# Autodesk Inventor assembly: A-01-0
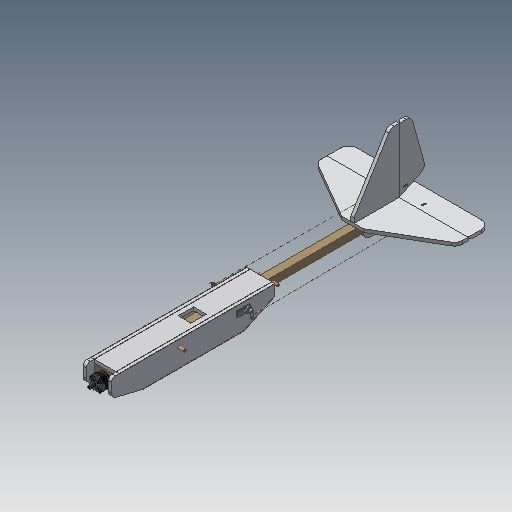
[picture p0: Inventor's stored thumbnail of the model, 512x512]
Saved by Autodesk Inventor 2019 (Build 230136000, 136)
## iProperties
Created: 2022-04-10
Part Number: A-01-0
Document SubType Name: Assembly
Designer: solyo
Mass: 82.8117 g
Surface Area: 1871.67 cm^2
Volume: 370.751 cm^3
Density: 0.223362 g/cm^3
Author: solyo
## Documents named in this file (19)
- D:\Modelling\RC\RC Trainer V1\ASSEMBLY\A-01-0-FUSELAGE\A-01-0.iam
- D:\Modelling\RC\RC Trainer V1\Parts\PW-00-0-TAILBOOM\PW-00-0-0.ipt
- D:\Modelling\RC\RC Trainer V1\Parts\PW-01-0-FIREWALL\PW-01-0-0.ipt
- D:\Modelling\RC\RC Trainer V1\Parts\PW-02-0-PIN\PW-02-0-0\WING_FRONT_TIE.ipt
- D:\Modelling\RC\RC Trainer V1\Design\Parts\PW-02-0-PIN\PW-02-0-0.ipt
- D:\Modelling\RC\RC Trainer V1\Parts\PW-02-0-PIN\PW-02-0-0\WING_REAR_TIE.ipt
- D:\Modelling\RC\RC Trainer V1\Parts\PF-01-0-FUSELAGE\PF-01-0-1.ipt
- D:\Modelling\RC\RC Trainer V1\Parts\C-01-0-EMAX_MT1806_2280KV\C-01-0.ipt
- D:\Modelling\RC\RC Trainer V1\Parts\PF-02-0-HORIZONTAL_STABILIZER\PF-02-0-0.ipt
- D:\Modelling\RC\RC Trainer V1\Parts\PF-03-0-VERTICAL_STABILIZER\PF-03-0-0.ipt
- D:\Modelling\RC\RC Trainer V1\Parts\PW-02-0-PIN\PW-02-0-0\SLIDE.ipt
- D:\Modelling\RC\RC Trainer V1\Parts\PM-00-0-PUSHROD\PM-00-0-0\TAIL.ipt
- D:\Modelling\RC\RC Trainer V1\Design\Parts\PM-00-0-PUSHROD\PM-00-0-0.ipt
- D:\Modelling\RC\RC Trainer V1\Parts\PP-00-0-CONTROL_HORN\PP-00-0-0.ipt
- D:\Modelling\RC\RC Trainer V1\Parts\C-02-0-EMAX_12AESC\C-02-0.ipt
- D:\Modelling\RC\RC Trainer V1\Parts\C-03-0-SERVO_3G\C-03-0\CW.ipt
- D:\Modelling\RC\RC Trainer V1\Design\Parts\C-03-0-SERVO_3G\C-03-0.ipt
- D:\Modelling\RC\RC Trainer V1\Parts\C-04-0-SERVO_LINKAGE_STOPPER\C-04-0.ipt
- D:\Modelling\RC\RC Trainer V1\Parts\C-05-0-FS2A_4CH\C-05-0.ipt
## Components (19 placed, 15 different names)
1. C-05-0:1 — Mate:39, Mate:40, Mate:41
2. PW-00-0-0:1
3. WING_FRONT_TIE:1
4. WING_REAR_TIE:2
5. C-02-0:1 — Mate:37, Flush:4, Mate:38
6. PW-01-0-0:1 — Flush:4, Mate:38, Mate:41
7. PF-01-0-1:1 — Flush:3, Mate:37, Mate:39, Mate:40
8. C-01-0:1
9. CW:1
10. CW:2
11. SLIDE:3
12. PF-02-0-0:1
13. PF-03-0-0:1
14. TAIL:1
15. TAIL:2
16. PP-00-0-0:1
17. PP-00-0-0:2
18. C-04-0:1
19. C-04-0:2
## Relationships (46: Mate 37, Insert 5, Flush 4)
- [Mate]: PW-00-0-0:1 ↔ PW-01-0-0:1
- [Flush]: PW-00-0-0:1 ↔ PW-01-0-0:1
- [Mate]: PW-00-0-0:1 ↔ PF-01-0-1:1
- [Mate]: PW-01-0-0:1 ↔ PF-01-0-1:1
- [Insert]: PW-01-0-0:1 ↔ C-01-0:1
- [Mate]: PW-01-0-0:1 ↔ C-01-0:1
- [Mate]: PF-02-0-0:1 ↔ PF-03-0-0:1
- [Mate]: PF-02-0-0:1 ↔ PF-03-0-0:1
- [Mate]: PF-02-0-0:1 ↔ PF-03-0-0:1
- [Mate]: PW-00-0-0:1 ↔ PF-03-0-0:1
- [Mate]: PW-00-0-0:1 ↔ PF-02-0-0:1
- [Mate]: PW-00-0-0:1 ↔ PF-03-0-0:1
- [Mate] (-2.5 mm): SLIDE:3 ↔ PF-03-0-0:1
- [Flush]: SLIDE:3 ↔ PF-03-0-0:1
- [Mate]: PF-02-0-0:1 ↔ PP-00-0-0:1
- [Mate]: PF-02-0-0:1 ↔ PP-00-0-0:1
- [Mate]: PF-03-0-0:1 ↔ PP-00-0-0:2
- [Mate]: PF-03-0-0:1 ↔ PP-00-0-0:2
- [Mate]: PW-00-0-0:1 ↔ CW:1
- [Mate]: PF-01-0-1:1 ↔ CW:1
- [Mate]: PW-00-0-0:1 ↔ CW:2
- [Mate]: PF-01-0-1:1 ↔ CW:2
- [Mate]: PF-01-0-1:1 ↔ CW:2
- [Mate] (10 mm): PF-02-0-0:1 ↔ PP-00-0-0:2
- [Mate]: PF-01-0-1:1 ↔ CW:1
- [Insert]: PP-00-0-0:2 ↔ C-04-0:1
- [Insert]: PP-00-0-0:1 ↔ C-04-0:2
- [Mate]: TAIL:1 ↔ C-04-0:2
- [Mate]: CW:2 ↔ TAIL:1
- [Mate] (1 mm): CW:2 ↔ TAIL:1
- [Insert] (-26 mm): PW-00-0-0:1 ↔ WING_FRONT_TIE:1
- [Mate]: WING_FRONT_TIE:1 ↔ PF-01-0-1:1
- [Insert] (-20 mm): PW-00-0-0:1 ↔ WING_REAR_TIE:2
- [Mate]: SLIDE:3 ↔ PF-03-0-0:1
- [Mate]: CW:1 ↔ TAIL:2
- [Mate] (1 mm): CW:1 ↔ TAIL:2
- [Mate]: TAIL:2 ↔ C-04-0:1
- [Mate]: CW:1 ↔ TAIL:2
- [Mate]: TAIL:2 ↔ C-04-0:1
- Flush:3: PF-01-0-1:1
- Mate:37: C-02-0:1 ↔ PF-01-0-1:1
- Flush:4: C-02-0:1 ↔ PW-01-0-0:1
- Mate:38 (10 mm): C-02-0:1 ↔ PW-01-0-0:1
- Mate:39: C-05-0:1 ↔ PF-01-0-1:1
- Mate:40: C-05-0:1 ↔ PF-01-0-1:1
- Mate:41 (15 mm): C-05-0:1 ↔ PW-01-0-0:1
## Named parameters: d37_d41 = 0 mm, d38_d42 = 0 mm
